# Autodesk Inventor assembly: Structure
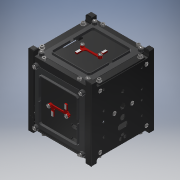
[picture p0: Inventor's stored thumbnail of the model, 180x180]
Saved by Autodesk Inventor 2018 (Build 220112000, 112)
## iProperties
Created: 2019-03-30
Part Number: Structure
Document SubType Name: Assembly
Designer: Bradley
Author: Bradley
## Documents named in this file (20)
- C:\Users\Bradley\Documents\GitHub\CougSat1-Hardware\CougSat1-Structure\CADModel\Imported\Structure.iam
- C:\Users\Bradley\Documents\GitHub\CougSat1-Hardware\CougSat1-Structure\CADModel\Imported\Structure_+X.ipt
- C:\Users\Bradley\Documents\GitHub\CougSat1-Hardware\CougSat1-Structure\CADModel\Imported\Structure_-X.ipt
- C:\Users\Bradley\Documents\GitHub\CougSat1-Hardware\CougSat1-Structure\CADModel\Imported\Structure_+Z.ipt
- C:\Users\Bradley\Documents\GitHub\CougSat1-Hardware\CougSat1-Structure\CADModel\Imported\Structure_Y.ipt
- C:\Users\Bradley\Documents\GitHub\CougSat1-Hardware\CougSat1-Structure\CADModel\Imported\Structure_-Z.ipt
- C:\Users\Bradley\Documents\GitHub\CougSat1-Hardware\CougSat1-Structure\CADModel\Imported\Structure_SolarPanelHeatsink.ipt
- C:\Users\Bradley\Documents\GitHub\CougSat1-Hardware\CougSat1-Structure\CADModel\Imported\Structure_MagnetorquerForm.ipt
- C:\Users\Bradley\Documents\GitHub\Resources\ComponentModels\Hardware\Spring_Separation.ipt
- C:\Users\Bradley\Documents\GitHub\Resources\ComponentModels\Fasteners\Bolt_M3x0.35_6mm_SH.ipt
- C:\Users\Bradley\Documents\GitHub\Resources\ComponentModels\Fasteners\Washer_3.2x7.0x0.6mm.ipt
- C:\Users\Bradley\Documents\GitHub\Resources\ComponentModels\Fasteners\Bolt_M3x0.35_5mm_SH.ipt
- C:\Users\Bradley\Documents\GitHub\Resources\ComponentModels\Fasteners\Bolt_M3x0.35_8mm_BH.ipt
- C:\Users\Bradley\Documents\GitHub\Resources\ComponentModels\Fasteners\Bolt_M3x0.35_4mm_BH.ipt
- C:\Users\Bradley\Documents\GitHub\Resources\ComponentModels\Fasteners\Bolt_M3x0.35_6mm_BH.ipt
- C:\Users\Bradley\Documents\GitHub\Resources\ComponentModels\Fasteners\Bolt_M3x0.35_10mm_BH.ipt
- C:\Users\Bradley\Documents\GitHub\Resources\ComponentModels\Electronics\Switch_Micro-Lever.iam
- C:\Users\Bradley\Documents\GitHub\Resources\ComponentModels\Fasteners\Bolt_M1.6x0.35_5mm_SH.ipt
- C:\Users\Bradley\Documents\GitHub\CougSat1-Hardware\CougSat1-Structure\CADModel\Imported\Structure_SwitchBlock.ipt
- C:\Users\Bradley\Documents\GitHub\CougSat1-Hardware\CougSat1-Structure\CADModel\Imported\Structure_SwitchPin.ipt
## Components (83 placed, 19 different names)
1. Structure_+X:1 — Mate:1, Mate:2, Insert:1, Insert:2, Mate:3, Insert:9, Insert:10, Insert:27, Insert:77, Insert:78, Insert:79, Insert:80, Insert:81, Insert:82
2. Structure_-X:1 — Insert:7, Insert:8, Insert:17, Insert:18, Insert:21, Insert:22, Insert:28, Insert:97, Insert:98, Insert:102, Angle:1
3. Structure_+Z:1 — Insert:1, Insert:2, Insert:3, Insert:4, Insert:5, Insert:6, Insert:7, Insert:8, Insert:13, Insert:14, Insert:23, Insert:24, Insert:30, Insert:38, Insert:41, Insert:42, Insert:43, Insert:44, Insert:45, Insert:46
4. Structure_Y:1 — Insert:3, Insert:4, Insert:11, Insert:12, Insert:19, Insert:20
5. Structure_Y:2 — Insert:5, Insert:6, Insert:15, Insert:16, Insert:25, Insert:26
6. Structure_-Z:1 — Insert:9, Insert:10, Insert:51, Insert:52, Insert:53, Insert:54, Insert:55, Insert:56, Insert:57, Insert:58, Insert:83, Insert:84, Insert:85, Insert:86
7. Structure_SolarPanelHeatsink:1 — Insert:13, Insert:14, Insert:73, Insert:74
8. Structure_SolarPanelHeatsink:2 — Insert:11, Insert:12, Insert:61, Insert:62
9. Structure_SolarPanelHeatsink:3 — Insert:17, Insert:18, Insert:95, Insert:96
10. Structure_SolarPanelHeatsink:4 — Insert:15, Insert:16, Insert:67, Insert:68
11. Structure_MagnetorquerForm:1 — Insert:19, Insert:20, Insert:59, Insert:60, Insert:63, Insert:64
12. Structure_MagnetorquerForm:2 — Insert:21, Insert:22, Insert:91, Insert:92, Insert:93, Insert:94
13. Structure_MagnetorquerForm:3 — Insert:23, Insert:24, Insert:71, Insert:72, Insert:75, Insert:76
14. Structure_MagnetorquerForm:4 — Insert:25, Insert:26, Insert:65, Insert:66, Insert:69, Insert:70
15. Spring_Separation:1 — Insert:27
16. Spring_Separation:2 — Insert:28
17. Bolt_M3x0.35_6mm_SH:1 — Insert:29
18. Washer_3.2x7.0x0.6mm:1 — Insert:29, Insert:30
19. Bolt_M3x0.35_5mm_SH:3 — Insert:45
20. Bolt_M3x0.35_5mm_SH:4 — Insert:46
21. Bolt_M3x0.35_6mm_SH:4
22. Washer_3.2x7.0x0.6mm:4 — Insert:41
23. Bolt_M3x0.35_6mm_SH:5
24. Washer_3.2x7.0x0.6mm:5 — Insert:42
25. Bolt_M3x0.35_5mm_SH:1 — Insert:43
26. Bolt_M3x0.35_5mm_SH:2 — Insert:44
27. Bolt_M3x0.35_6mm_SH:8
28. Washer_3.2x7.0x0.6mm:8 — Insert:38
29. Bolt_M3x0.35_6mm_SH:9
30. Washer_3.2x7.0x0.6mm:9 — Insert:54
31. Bolt_M3x0.35_6mm_SH:10
32. Washer_3.2x7.0x0.6mm:10 — Insert:53
33. Bolt_M3x0.35_6mm_SH:11
34. Washer_3.2x7.0x0.6mm:11 — Insert:51
35. Bolt_M3x0.35_6mm_SH:12
36. Washer_3.2x7.0x0.6mm:12 — Insert:52
37. Bolt_M3x0.35_5mm_SH:5 — Insert:58
38. Bolt_M3x0.35_5mm_SH:6 — Insert:57
39. Bolt_M3x0.35_5mm_SH:7 — Insert:55
40. Bolt_M3x0.35_5mm_SH:8 — Insert:56
41. Bolt_M3x0.35_8mm_BH:1 — Insert:59
42. Bolt_M3x0.35_8mm_BH:2 — Insert:60
43. Bolt_M3x0.35_8mm_BH:3 — Insert:63
44. Bolt_M3x0.35_8mm_BH:4 — Insert:64
45. Bolt_M3x0.35_8mm_BH:5 — Insert:61
46. Bolt_M3x0.35_8mm_BH:6 — Insert:62
47. Bolt_M3x0.35_8mm_BH:7 — Insert:65
48. Bolt_M3x0.35_8mm_BH:8 — Insert:66
49. Bolt_M3x0.35_8mm_BH:9 — Insert:67
50. Bolt_M3x0.35_8mm_BH:10 — Insert:68
51. Bolt_M3x0.35_8mm_BH:11 — Insert:69
52. Bolt_M3x0.35_8mm_BH:12 — Insert:70
53. Bolt_M3x0.35_8mm_BH:13 — Insert:71
54. Bolt_M3x0.35_8mm_BH:14 — Insert:72
55. Bolt_M3x0.35_8mm_BH:15 — Insert:74
56. Bolt_M3x0.35_8mm_BH:16 — Insert:73
57. Bolt_M3x0.35_8mm_BH:17 — Insert:76
58. Bolt_M3x0.35_8mm_BH:18 — Insert:75
59. Bolt_M3x0.35_4mm_BH:1 — Insert:77
60. Bolt_M3x0.35_4mm_BH:2 — Insert:78
61. Bolt_M3x0.35_4mm_BH:3 — Insert:79
62. Bolt_M3x0.35_4mm_BH:4 — Insert:80
63. Bolt_M3x0.35_4mm_BH:5 — Insert:81
64. Bolt_M3x0.35_4mm_BH:6 — Insert:82
65. Washer_3.2x7.0x0.6mm:13 — Insert:83, Insert:87
66. Washer_3.2x7.0x0.6mm:14 — Insert:84, Insert:88
67. Washer_3.2x7.0x0.6mm:15 — Insert:85, Insert:90
68. Washer_3.2x7.0x0.6mm:16 — Insert:86, Insert:89
69. Bolt_M3x0.35_4mm_BH:7 — Insert:87
70. Bolt_M3x0.35_4mm_BH:8 — Insert:88
71. Bolt_M3x0.35_4mm_BH:9 — Insert:90
72. Bolt_M3x0.35_4mm_BH:10 — Insert:89
73. Bolt_M3x0.35_6mm_BH:1 — Insert:91
74. Bolt_M3x0.35_6mm_BH:2 — Insert:92
75. Bolt_M3x0.35_6mm_BH:3 — Insert:94
76. Bolt_M3x0.35_6mm_BH:4 — Insert:93
77. Bolt_M3x0.35_10mm_BH:1 — Insert:95
78. Bolt_M3x0.35_10mm_BH:2 — Insert:96
79. Switch_Micro-Lever:1 [sub-assembly] — Insert:97, Insert:98, Insert:99, Insert:100
80. Bolt_M1.6x0.35_5mm_SH:1 — Insert:100
81. Bolt_M1.6x0.35_5mm_SH:2 — Insert:99
82. Structure_SwitchBlock:1 — Insert:101, Angle:1
83. Structure_SwitchPin:1 — Insert:101, Insert:102
## Relationships (100: Insert 96, Mate 3, Angle 1)
- Mate:1 (50 mm): Structure_+X:1
- Mate:2 (-49 mm): Structure_+X:1
- Insert:1: Structure_+X:1 ↔ Structure_+Z:1
- Insert:2: Structure_+X:1 ↔ Structure_+Z:1
- Insert:3: Structure_+Z:1 ↔ Structure_Y:1
- Insert:4: Structure_+Z:1 ↔ Structure_Y:1
- Insert:5: Structure_+Z:1 ↔ Structure_Y:2
- Insert:6: Structure_+Z:1 ↔ Structure_Y:2
- Insert:7: Structure_-X:1 ↔ Structure_+Z:1
- Insert:8: Structure_-X:1 ↔ Structure_+Z:1
- Mate:3 (50 mm): Structure_+X:1
- Insert:9: Structure_+X:1 ↔ Structure_-Z:1
- Insert:10: Structure_+X:1 ↔ Structure_-Z:1
- Insert:11: Structure_Y:1 ↔ Structure_SolarPanelHeatsink:2
- Insert:12: Structure_Y:1 ↔ Structure_SolarPanelHeatsink:2
- Insert:13: Structure_+Z:1 ↔ Structure_SolarPanelHeatsink:1
- Insert:14: Structure_+Z:1 ↔ Structure_SolarPanelHeatsink:1
- Insert:15: Structure_Y:2 ↔ Structure_SolarPanelHeatsink:4
- Insert:16: Structure_Y:2 ↔ Structure_SolarPanelHeatsink:4
- Insert:17: Structure_-X:1 ↔ Structure_SolarPanelHeatsink:3
- Insert:18: Structure_-X:1 ↔ Structure_SolarPanelHeatsink:3
- Insert:19: Structure_Y:1 ↔ Structure_MagnetorquerForm:1
- Insert:20: Structure_Y:1 ↔ Structure_MagnetorquerForm:1
- Insert:21: Structure_-X:1 ↔ Structure_MagnetorquerForm:2
- Insert:22: Structure_-X:1 ↔ Structure_MagnetorquerForm:2
- Insert:23: Structure_+Z:1 ↔ Structure_MagnetorquerForm:3
- Insert:24: Structure_+Z:1 ↔ Structure_MagnetorquerForm:3
- Insert:25: Structure_Y:2 ↔ Structure_MagnetorquerForm:4
- Insert:26: Structure_Y:2 ↔ Structure_MagnetorquerForm:4
- Insert:27: Structure_+X:1 ↔ Spring_Separation:1
- Insert:28: Structure_-X:1 ↔ Spring_Separation:2
- Insert:29: Bolt_M3x0.35_6mm_SH:1 ↔ Washer_3.2x7.0x0.6mm:1
- Insert:30: Structure_+Z:1 ↔ Washer_3.2x7.0x0.6mm:1
- [Insert]: Bolt_M3x0.35_6mm_SH:4 ↔ Washer_3.2x7.0x0.6mm:4
- [Insert]: Bolt_M3x0.35_6mm_SH:5 ↔ Washer_3.2x7.0x0.6mm:5
- [Insert]: Bolt_M3x0.35_6mm_SH:8 ↔ Washer_3.2x7.0x0.6mm:8
- Insert:38: Structure_+Z:1 ↔ Washer_3.2x7.0x0.6mm:8
- Insert:41: Structure_+Z:1 ↔ Washer_3.2x7.0x0.6mm:4
- Insert:42: Structure_+Z:1 ↔ Washer_3.2x7.0x0.6mm:5
- Insert:43: Structure_+Z:1 ↔ Bolt_M3x0.35_5mm_SH:1
- Insert:44: Structure_+Z:1 ↔ Bolt_M3x0.35_5mm_SH:2
- Insert:45: Structure_+Z:1 ↔ Bolt_M3x0.35_5mm_SH:3
- Insert:46: Structure_+Z:1 ↔ Bolt_M3x0.35_5mm_SH:4
- [Insert]: Bolt_M3x0.35_6mm_SH:9 ↔ Washer_3.2x7.0x0.6mm:9
- [Insert]: Bolt_M3x0.35_6mm_SH:10 ↔ Washer_3.2x7.0x0.6mm:10
- [Insert]: Bolt_M3x0.35_6mm_SH:11 ↔ Washer_3.2x7.0x0.6mm:11
- [Insert]: Bolt_M3x0.35_6mm_SH:12 ↔ Washer_3.2x7.0x0.6mm:12
- Insert:51: Structure_-Z:1 ↔ Washer_3.2x7.0x0.6mm:11
- Insert:52: Structure_-Z:1 ↔ Washer_3.2x7.0x0.6mm:12
- Insert:53: Structure_-Z:1 ↔ Washer_3.2x7.0x0.6mm:10
- Insert:54: Structure_-Z:1 ↔ Washer_3.2x7.0x0.6mm:9
- Insert:55: Structure_-Z:1 ↔ Bolt_M3x0.35_5mm_SH:7
- Insert:56: Structure_-Z:1 ↔ Bolt_M3x0.35_5mm_SH:8
- Insert:57: Structure_-Z:1 ↔ Bolt_M3x0.35_5mm_SH:6
- Insert:58: Structure_-Z:1 ↔ Bolt_M3x0.35_5mm_SH:5
- Insert:59 (0.6 mm): Structure_MagnetorquerForm:1 ↔ Bolt_M3x0.35_8mm_BH:1
- Insert:60 (0.6 mm): Structure_MagnetorquerForm:1 ↔ Bolt_M3x0.35_8mm_BH:2
- Insert:61 (0.6 mm): Structure_SolarPanelHeatsink:2 ↔ Bolt_M3x0.35_8mm_BH:5
- Insert:62 (0.6 mm): Structure_SolarPanelHeatsink:2 ↔ Bolt_M3x0.35_8mm_BH:6
- Insert:63 (0.6 mm): Structure_MagnetorquerForm:1 ↔ Bolt_M3x0.35_8mm_BH:3
- Insert:64 (0.6 mm): Structure_MagnetorquerForm:1 ↔ Bolt_M3x0.35_8mm_BH:4
- Insert:65 (0.6 mm): Structure_MagnetorquerForm:4 ↔ Bolt_M3x0.35_8mm_BH:7
- Insert:66 (0.6 mm): Structure_MagnetorquerForm:4 ↔ Bolt_M3x0.35_8mm_BH:8
- Insert:67 (0.6 mm): Structure_SolarPanelHeatsink:4 ↔ Bolt_M3x0.35_8mm_BH:9
- Insert:68 (0.6 mm): Structure_SolarPanelHeatsink:4 ↔ Bolt_M3x0.35_8mm_BH:10
- Insert:69 (0.6 mm): Structure_MagnetorquerForm:4 ↔ Bolt_M3x0.35_8mm_BH:11
- Insert:70 (0.6 mm): Structure_MagnetorquerForm:4 ↔ Bolt_M3x0.35_8mm_BH:12
- Insert:71 (0.6 mm): Structure_MagnetorquerForm:3 ↔ Bolt_M3x0.35_8mm_BH:13
- Insert:72 (0.6 mm): Structure_MagnetorquerForm:3 ↔ Bolt_M3x0.35_8mm_BH:14
- Insert:73 (0.6 mm): Structure_SolarPanelHeatsink:1 ↔ Bolt_M3x0.35_8mm_BH:16
- Insert:74 (0.6 mm): Structure_SolarPanelHeatsink:1 ↔ Bolt_M3x0.35_8mm_BH:15
- Insert:75 (0.6 mm): Structure_MagnetorquerForm:3 ↔ Bolt_M3x0.35_8mm_BH:18
- Insert:76 (0.6 mm): Structure_MagnetorquerForm:3 ↔ Bolt_M3x0.35_8mm_BH:17
- Insert:77 (0.6 mm): Structure_+X:1 ↔ Bolt_M3x0.35_4mm_BH:1
- Insert:78 (0.6 mm): Structure_+X:1 ↔ Bolt_M3x0.35_4mm_BH:2
- Insert:79 (0.6 mm): Structure_+X:1 ↔ Bolt_M3x0.35_4mm_BH:3
- Insert:80 (0.6 mm): Structure_+X:1 ↔ Bolt_M3x0.35_4mm_BH:4
- Insert:81 (0.6 mm): Structure_+X:1 ↔ Bolt_M3x0.35_4mm_BH:5
- Insert:82 (0.6 mm): Structure_+X:1 ↔ Bolt_M3x0.35_4mm_BH:6
- Insert:83: Structure_-Z:1 ↔ Washer_3.2x7.0x0.6mm:13
- Insert:84: Structure_-Z:1 ↔ Washer_3.2x7.0x0.6mm:14
- Insert:85: Structure_-Z:1 ↔ Washer_3.2x7.0x0.6mm:15
- Insert:86: Structure_-Z:1 ↔ Washer_3.2x7.0x0.6mm:16
- Insert:87 (0.6 mm): Washer_3.2x7.0x0.6mm:13 ↔ Bolt_M3x0.35_4mm_BH:7
- Insert:88 (0.6 mm): Washer_3.2x7.0x0.6mm:14 ↔ Bolt_M3x0.35_4mm_BH:8
- Insert:89 (0.6 mm): Washer_3.2x7.0x0.6mm:16 ↔ Bolt_M3x0.35_4mm_BH:10
- Insert:90 (0.6 mm): Washer_3.2x7.0x0.6mm:15 ↔ Bolt_M3x0.35_4mm_BH:9
- Insert:91 (0.6 mm): Structure_MagnetorquerForm:2 ↔ Bolt_M3x0.35_6mm_BH:1
- Insert:92 (0.6 mm): Structure_MagnetorquerForm:2 ↔ Bolt_M3x0.35_6mm_BH:2
- Insert:93 (0.6 mm): Structure_MagnetorquerForm:2 ↔ Bolt_M3x0.35_6mm_BH:4
- Insert:94 (0.6 mm): Structure_MagnetorquerForm:2 ↔ Bolt_M3x0.35_6mm_BH:3
- Insert:95 (0.6 mm): Structure_SolarPanelHeatsink:3 ↔ Bolt_M3x0.35_10mm_BH:1
- Insert:96 (0.6 mm): Structure_SolarPanelHeatsink:3 ↔ Bolt_M3x0.35_10mm_BH:2
- Insert:97: Structure_-X:1 ↔ Switch_Micro-Lever:1
- Insert:98: Structure_-X:1 ↔ Switch_Micro-Lever:1
- Insert:99: Switch_Micro-Lever:1 ↔ Bolt_M1.6x0.35_5mm_SH:2
- Insert:100: Switch_Micro-Lever:1 ↔ Bolt_M1.6x0.35_5mm_SH:1
- Insert:101: Structure_SwitchBlock:1 ↔ Structure_SwitchPin:1
- Insert:102 (-0.75 mm): Structure_-X:1 ↔ Structure_SwitchPin:1
- Angle:1 (0 deg): Structure_-X:1 ↔ Structure_SwitchBlock:1
## Named parameters: d36_d32 = 0 mm, d37_d32 = 0 mm, d40_d32 = 0 mm, d52_d32 = 0 mm, d53_d32 = 0 mm, d54_d32 = 0 mm, d55_d32 = 0 mm, SolarPanelThickness = 0.6 mm, PXThickness = 0.6 mm, NZThickness = 0.6 mm
